# Autodesk Inventor assembly: Water Table 4x4 v2
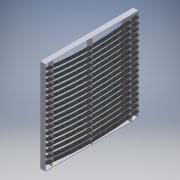
[picture p0: Inventor's stored thumbnail of the model, 180x180]
Saved by Autodesk Inventor 2019 (Build 230136000, 136)
## iProperties
Created: 2017-12-19
Part Number: Water Table 4x4 v2
Document SubType Name: Assembly
Designer: torba
Author: torba
## Documents named in this file (10)
- C:\Users\torba\Nextcloud\Projects\Inventor\Plasma 5x10\Water Table 4x4 v2.iam
- C:\Users\torba\OneDrive\Documents\Inventor\Plasma 5x10\3 x 3 angle 45 .25 steel.ipt
- C:\Users\torba\OneDrive\Documents\Inventor\Plasma 5x10\1-16 sheet metal.ipt
- C:\Users\torba\Nextcloud\Projects\Inventor\Plasma 5x10\1-16 sheet metal\1-16 sheet metal-48x48.ipt
- C:\Users\torba\Nextcloud\Projects\Inventor\Plasma 5x10\3 x 3 angle 45 .25 steel\3 x 3 angle 45 .25 steel-54.ipt
- C:\Users\torba\Nextcloud\Projects\Inventor\Plasma 5x10\3 x 3.25 steel side slit\3 x 3 angle 45 .25 steel-54.ipt
- C:\Users\torba\OneDrive\Documents\Inventor\Plasma 5x10\3 x 3.25 steel side slit.ipt
- C:\Users\torba\Nextcloud\Projects\Inventor\Plasma 5x10\3 x 3.25 steel side slit center\3 x 3 angle 45 .25 steel-54.ipt
- C:\Users\torba\OneDrive\Documents\Inventor\Plasma 5x10\3 x 3.25 steel side slit center.ipt
- C:\Users\torba\Nextcloud\Projects\Inventor\Plasma 5x10\bent slat v2.ipt
## Components (9 placed, 3 different names)
1. 3 x 3 angle 45 .25 steel-54:1 — Flush:2, Mate:3, Mate:4, Flush:3, Mate:6, Mate:27
2. 3 x 3 angle 45 .25 steel-54:2 — Mate:1, Flush:1, Mate:2, Mate:5, Flush:4, Mate:10, Mate:23, Mate:28, Mate:30
3. 3 x 3 angle 45 .25 steel-54:3 — Mate:1, Flush:1, Mate:2, Flush:2, Mate:3, Mate:4, Mate:13, Mate:18, Mate:19
4. 3 x 3 angle 45 .25 steel-54:4 — Flush:3, Mate:5, Mate:6, Mate:11, Mate:15, Mate:21, Mate:22
5. 1-16 sheet metal-48x48:1 — Flush:4, Mate:10, Mate:11
6. 3 x 3 angle 45 .25 steel-54:1 — Mate:21, Mate:22, Mate:23, Mate:31
7. 3 x 3 angle 45 .25 steel-54:2 — Mate:18, Mate:19, Mate:28
8. 3 x 3 angle 45 .25 steel-54:3 — Mate:13, Mate:15, Mate:27, Mate:29
9. bent slat v2:1 — Mate:29, Mate:30, Mate:31
## Relationships (24: Mate 20, Flush 4)
- Mate:1: 3 x 3 angle 45 .25 steel-54:2 ↔ 3 x 3 angle 45 .25 steel-54:3
- Flush:1: 3 x 3 angle 45 .25 steel-54:2 ↔ 3 x 3 angle 45 .25 steel-54:3
- Mate:2: 3 x 3 angle 45 .25 steel-54:2 ↔ 3 x 3 angle 45 .25 steel-54:3
- Flush:2: 3 x 3 angle 45 .25 steel-54:1 ↔ 3 x 3 angle 45 .25 steel-54:3
- Mate:3: 3 x 3 angle 45 .25 steel-54:1 ↔ 3 x 3 angle 45 .25 steel-54:3
- Mate:4: 3 x 3 angle 45 .25 steel-54:1 ↔ 3 x 3 angle 45 .25 steel-54:3
- Flush:3: 3 x 3 angle 45 .25 steel-54:1 ↔ 3 x 3 angle 45 .25 steel-54:4
- Mate:5: 3 x 3 angle 45 .25 steel-54:2 ↔ 3 x 3 angle 45 .25 steel-54:4
- Mate:6: 3 x 3 angle 45 .25 steel-54:1 ↔ 3 x 3 angle 45 .25 steel-54:4
- Flush:4: 3 x 3 angle 45 .25 steel-54:2 ↔ 1-16 sheet metal-48x48:1
- Mate:10: 3 x 3 angle 45 .25 steel-54:2 ↔ 1-16 sheet metal-48x48:1
- Mate:11: 3 x 3 angle 45 .25 steel-54:4 ↔ 1-16 sheet metal-48x48:1
- Mate:13: 3 x 3 angle 45 .25 steel-54:3
- Mate:15: 3 x 3 angle 45 .25 steel-54:4 ↔ 3 x 3 angle 45 .25 steel-54:3
- Mate:18: 3 x 3 angle 45 .25 steel-54:3 ↔ 3 x 3 angle 45 .25 steel-54:2
- Mate:19: 3 x 3 angle 45 .25 steel-54:3 ↔ 3 x 3 angle 45 .25 steel-54:2
- Mate:21: 3 x 3 angle 45 .25 steel-54:4 ↔ 3 x 3 angle 45 .25 steel-54:1
- Mate:22: 3 x 3 angle 45 .25 steel-54:4 ↔ 3 x 3 angle 45 .25 steel-54:1
- Mate:23 (676.275 mm): 3 x 3 angle 45 .25 steel-54:2 ↔ 3 x 3 angle 45 .25 steel-54:1
- Mate:27 (101.6 mm): 3 x 3 angle 45 .25 steel-54:1 ↔ 3 x 3 angle 45 .25 steel-54:3
- Mate:28 (101.6 mm): 3 x 3 angle 45 .25 steel-54:2
- Mate:29: 3 x 3 angle 45 .25 steel-54:3 ↔ bent slat v2:1
- Mate:30: 3 x 3 angle 45 .25 steel-54:2 ↔ bent slat v2:1
- Mate:31: 3 x 3 angle 45 .25 steel-54:1 ↔ bent slat v2:1
